# Autodesk Inventor assembly: MG-Chip Kicker
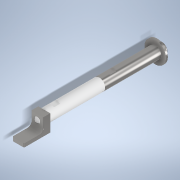
[picture p0: Inventor's stored thumbnail of the model, 180x180]
Saved by Autodesk Inventor 2020 (Build 240168000, 168)
## iProperties
Part Number: MG-Chip Kicker
Material: Generisch
Document SubType Name: Assembly
Designer: rYan
Mass: 43.8833 g
Surface Area: 57.8442 cm^2
Volume: 9.33315 cm^3
Density: 4.70187 g/cm^3
Author: rYan
## Documents named in this file (6)
- D:\github\ssl-mechanics\V2.1(LARC2019)\Inventor\kicker\kicker_assembly_chip.iam
- D:\github\ssl-mechanics\V2.1(LARC2019)\Inventor\kicker\kicker_mitte.ipt
- D:\github\ssl-mechanics\V2.1(LARC2019)\Inventor\kicker\kicker_eisen.ipt
- D:\github\ssl-mechanics\V2.1(LARC2019)\Inventor\kicker\kicker_chip_head.ipt
- D:\github\ssl-mechanics\V2.1(LARC2019)\Inventor\kicker\compras\DIN 9021 - 6,4.ipt
- D:\github\ssl-mechanics\V2.1(LARC2019)\Inventor\kicker\compras\DIN 7984 - M6 x 10.ipt
## Components (5 placed, 4 different names)
1. Kicker Eisen:1 — Einfügen:1, Einfügen:2, Fluchtend:1
2. Kicker Eisen:1 — Einfügen:1, Einfügen:4
3. Kicker Chip Head:1 — Einfügen:2, Fluchtend:1
4. DIN 9021 6,4:1 — Einfügen:4
5. DIN 7984 M6 x 10:1
## Relationships (5: Insert 4, Flush 1)
- Einfügen:1 [Insert]: Kicker Eisen:1
- Einfügen:2 [Insert]: Kicker Eisen:1 ↔ Kicker Chip Head:1
- Fluchtend:1 [Flush]: Kicker Eisen:1 ↔ Kicker Chip Head:1
- [Insert]: DIN 9021 6,4:1 ↔ DIN 7984 M6 x 10:1
- Einfügen:4 [Insert]: Kicker Eisen:1 ↔ DIN 9021 6,4:1
